# Autodesk Inventor assembly: OBG-Elektronik
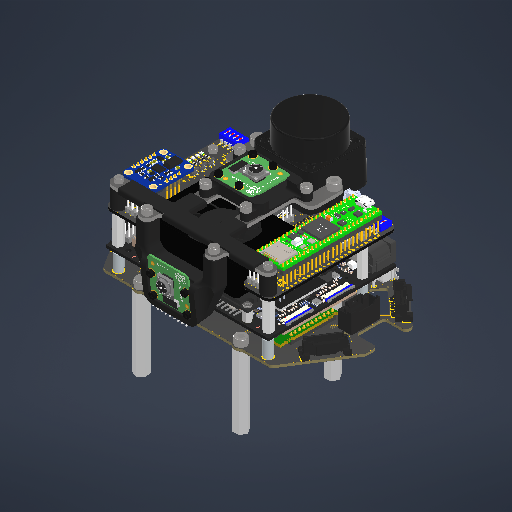
[picture p0: Inventor's stored thumbnail of the model, 512x512]
Saved by Autodesk Inventor 2025.2 (Build 292293000, 293)
## iProperties
Created: 2024-11-26
Part Number: OBG-Elektronik
Document SubType Name: Assembly
Designer: Fabian
Author: Fabian
## Documents named in this file (19)
- C:\Users\Faabs\Desktop\HBG v2025\Oberbaugruppen\OBG-Elektronik\OBG-Elektronik.iam
- C:\Users\Faabs\Desktop\HBG v2025\Oberbaugruppen\OBG-Elektronik\Bauteile\Abstandsbolzen 45mm.ipt
- C:\Users\Faabs\Desktop\HBG v2025\Oberbaugruppen\OBG-Elektronik\Bauteile\Jetson Orin Nano\Jetson Orin Nano.iam
- C:\Users\Faabs\Desktop\HBG v2025\Oberbaugruppen\OBG-Elektronik\Bauteile\Abstandsbolzen 17mm.ipt
- C:\Users\Faabs\Desktop\HBG v2025\Oberbaugruppen\OBG-Elektronik\Bauteile\360° LiDAR\360° LiDAR.iam
- C:\Users\Faabs\Desktop\HBG v2025\Verbindungselemente\DIN 912\DIN 912 - M4 x 0,7 x 8 x 6,25.ipt
- C:\Users\Faabs\Desktop\HBG v2025\Verbindungselemente\DIN 912\DIN 912 - M2,5 x 0,45 x 8 x 6,875.ipt
- C:\Users\Faabs\Desktop\HBG v2025\Oberbaugruppen\OBG-Elektronik\Bauteile\Trägerblech.ipt
- C:\Users\Faabs\Desktop\HBG v2025\Oberbaugruppen\OBG-Elektronik\Bauteile\Kamera.ipt
- C:\Users\Faabs\Desktop\HBG v2025\Oberbaugruppen\OBG-Elektronik\Bauteile\Kamerahalterung oben.ipt
- C:\Users\Faabs\Desktop\HBG v2025\Verbindungselemente\DIN 912\DIN 912 - M3 x 0,5 x 5 x 3,75.ipt
- C:\Users\Faabs\Desktop\HBG v2025\Oberbaugruppen\OBG-Elektronik\Bauteile\Abstandshalter 11mm.ipt
- C:\Users\Faabs\Desktop\HBG v2025\Oberbaugruppen\OBG-Elektronik\Bauteile\Abstandshalter 7,4mm.ipt
- C:\Users\Faabs\Desktop\HBG v2025\Verbindungselemente\DIN 912\DIN 912 - M4 x 0,7 x 16 x 14,25.ipt
- C:\Users\Faabs\Desktop\HBG v2025\Platinen\Steuerplatine\Steuerplatine\Steuerplatine.iam
- C:\Users\Faabs\Desktop\HBG v2025\Platinen\Hauptplatine\HauptplatineV2\HauptplatineV2.iam
- C:\Users\Faabs\Desktop\HBG v2025\Oberbaugruppen\OBG-Elektronik\Bauteile\Spiegelflächenabdeckung.ipt
- C:\Users\Faabs\Desktop\HBG v2025\Oberbaugruppen\OBG-Elektronik\Bauteile\Kamerahalterung vorne.ipt
- C:\Users\Faabs\Desktop\HBG v2025\Verbindungselemente\DIN 912\DIN 912 - M2 x 0,4 x 4 x 3.ipt
## Components (46 placed, 18 different names)
1. Jetson Orin Nano:1 [sub-assembly] — Passend:14, Passend:15, Passend:16, Passend:17, Passend:18, Passend:19, Passend:20, Passend:21, Passend:76
2. Steuerplatine:1 [sub-assembly] — Einfügen:27, Einfügen:29, Einfügen:30, Einfügen:35, Einfügen:36, Passend:79, Passend:80, Passend:82, Passend:83
3. HauptplatineV2:1 [sub-assembly] — Passend:64, Fluchtend:1, Passend:74, Passend:75, Passend:76, Passend:106, Passend:107, Passend:108, Passend:109, Passend:110, Passend:111, Passend:112, Passend:113, Einfügen:44, Einfügen:45, Einfügen:46, Einfügen:47
4. 360° LiDAR:1 [sub-assembly] — Passend:48, Passend:49, Passend:50, Passend:51, Einfügen:29, Einfügen:30
5. DIN 912 - ersetzt durch DIN EN ISO 4762 M2 x 4:8 — Einfügen:52
6. DIN 912 - ersetzt durch DIN EN ISO 4762 M2 x 4:7 — Einfügen:53
7. DIN 912 - ersetzt durch DIN EN ISO 4762 M2 x 4:6 — Einfügen:54
8. DIN 912 - ersetzt durch DIN EN ISO 4762 M2 x 4:5 — Einfügen:55
9. DIN 912 - ersetzt durch DIN EN ISO 4762 M2 x 4:4 — Einfügen:51
10. DIN 912 - ersetzt durch DIN EN ISO 4762 M2 x 4:3 — Einfügen:49
11. DIN 912 - ersetzt durch DIN EN ISO 4762 M2 x 4:2 — Einfügen:50
12. DIN 912 - ersetzt durch DIN EN ISO 4762 M2 x 4:1 — Einfügen:48
13. DIN 912 - ersetzt durch DIN EN ISO 4762 M3 x 5:6 — Einfügen:42
14. DIN 912 - ersetzt durch DIN EN ISO 4762 M3 x 5:5 — Einfügen:41, Passend:102
15. DIN 912 - ersetzt durch DIN EN ISO 4762 M4 x 16:2 — Einfügen:18
16. DIN 912 - ersetzt durch DIN EN ISO 4762 M4 x 16:1 — Einfügen:17
17. DIN 912 - ersetzt durch DIN EN ISO 4762 M3 x 5:4 — Einfügen:11
18. DIN 912 - ersetzt durch DIN EN ISO 4762 M3 x 5:3 — Einfügen:12
19. DIN 912 - ersetzt durch DIN EN ISO 4762 M3 x 5:2 — Einfügen:13
20. DIN 912 - ersetzt durch DIN EN ISO 4762 M3 x 5:1 — Einfügen:14
21. DIN 912 - ersetzt durch DIN EN ISO 4762 M4 x 8:1 — Einfügen:44
22. DIN 912 - ersetzt durch DIN EN ISO 4762 M4 x 8:2 — Einfügen:45
23. DIN 912 - ersetzt durch DIN EN ISO 4762 M4 x 8:3 — Einfügen:47
24. DIN 912 - ersetzt durch DIN EN ISO 4762 M4 x 8:4 — Einfügen:46
25. DIN 912 - ersetzt durch DIN EN ISO 4762 M2,5 x 8:1 — Einfügen:39
26. DIN 912 - ersetzt durch DIN EN ISO 4762 M2,5 x 8:2 — Einfügen:35, Passend:81
27. DIN 912 - ersetzt durch DIN EN ISO 4762 M2,5 x 8:3 — Einfügen:40
28. DIN 912 - ersetzt durch DIN EN ISO 4762 M2,5 x 8:4 — Einfügen:36
29. Abstandshalter 11mm:1 — Passend:82, Passend:83, Passend:85
30. Abstandshalter 11mm:2 — Einfügen:27, Passend:84
31. Abstandshalter 7,4mm:1 — Passend:49, Passend:50, Passend:63
32. Abstandshalter 7,4mm:2 — Passend:48, Passend:51
33. Abstandsbolzen 45mm:1 — Passend:108, Passend:113
34. Abstandsbolzen 45mm:2 — Passend:109, Passend:110
35. Abstandsbolzen 45mm:3 — Passend:106, Passend:111, Passend:114
36. Abstandsbolzen 45mm:4 — Passend:107, Passend:112
37. Abstandsbolzen 17mm:1 — Passend:14, Passend:21, Passend:79, Passend:80
38. Abstandsbolzen 17mm:2 — Passend:15, Passend:18, Passend:75
39. Abstandsbolzen 17mm:3 — Passend:16, Passend:20, Passend:74
40. Abstandsbolzen 17mm:4 — Passend:17, Passend:19, Passend:81
41. Kamera:3 — Passend:103, Passend:104, Passend:105, Einfügen:52, Einfügen:53, Einfügen:54, Einfügen:55
42. Kamerahalterung vorne:1 — Einfügen:43, Passend:102, Passend:103, Passend:104, Passend:105
43. Spiegelflächenabdeckung:1 — Passend:98, Passend:99, Passend:100
44. Trägerblech:1 — Passend:38, Einfügen:17, Einfügen:18, Passend:63, Einfügen:37, Einfügen:38, Passend:84, Passend:85, Einfügen:39, Einfügen:40, Passend:98, Passend:99, Passend:100, Einfügen:41, Einfügen:42, Einfügen:43
45. Kamera:1 — Passend:39, Passend:40, Passend:41, Einfügen:48, Einfügen:49, Einfügen:50, Einfügen:51
46. Kamerahalterung oben:1 — Passend:38, Passend:39, Passend:40, Passend:41, Einfügen:11, Einfügen:12, Einfügen:13, Einfügen:14, Einfügen:37, Einfügen:38
## Relationships (75: Mate 44, Insert 30, Flush 1)
- Passend:14 [Mate]: Jetson Orin Nano:1 ↔ Abstandsbolzen 17mm:1
- Passend:15 [Mate]: Jetson Orin Nano:1 ↔ Abstandsbolzen 17mm:2
- Passend:16 [Mate]: Jetson Orin Nano:1 ↔ Abstandsbolzen 17mm:3
- Passend:17 [Mate]: Jetson Orin Nano:1 ↔ Abstandsbolzen 17mm:4
- Passend:18 [Mate]: Jetson Orin Nano:1 ↔ Abstandsbolzen 17mm:2
- Passend:19 [Mate]: Jetson Orin Nano:1 ↔ Abstandsbolzen 17mm:4
- Passend:20 [Mate]: Jetson Orin Nano:1 ↔ Abstandsbolzen 17mm:3
- Passend:21 [Mate]: Jetson Orin Nano:1 ↔ Abstandsbolzen 17mm:1
- Passend:38 [Mate]: Trägerblech:1 ↔ Kamerahalterung oben:1
- Passend:39 [Mate]: Kamera:1 ↔ Kamerahalterung oben:1
- Passend:40 [Mate]: Kamera:1 ↔ Kamerahalterung oben:1
- Passend:41 [Mate]: Kamera:1 ↔ Kamerahalterung oben:1
- Einfügen:11 [Insert]: DIN 912 - ersetzt durch DIN EN ISO 4762 M3 x 5:4 ↔ Kamerahalterung oben:1
- Einfügen:12 [Insert]: DIN 912 - ersetzt durch DIN EN ISO 4762 M3 x 5:3 ↔ Kamerahalterung oben:1
- Einfügen:13 [Insert]: DIN 912 - ersetzt durch DIN EN ISO 4762 M3 x 5:2 ↔ Kamerahalterung oben:1
- Einfügen:14 [Insert]: DIN 912 - ersetzt durch DIN EN ISO 4762 M3 x 5:1 ↔ Kamerahalterung oben:1
- Passend:48 [Mate]: 360° LiDAR:1 ↔ Abstandshalter 7,4mm:2
- Passend:49 [Mate]: 360° LiDAR:1 ↔ Abstandshalter 7,4mm:1
- Passend:50 [Mate]: 360° LiDAR:1 ↔ Abstandshalter 7,4mm:1
- Passend:51 [Mate]: 360° LiDAR:1 ↔ Abstandshalter 7,4mm:2
- Einfügen:17 [Insert]: DIN 912 - ersetzt durch DIN EN ISO 4762 M4 x 16:1 ↔ Trägerblech:1
- Einfügen:18 [Insert]: DIN 912 - ersetzt durch DIN EN ISO 4762 M4 x 16:2 ↔ Trägerblech:1
- Einfügen:27 [Insert]: Steuerplatine:1 ↔ Abstandshalter 11mm:2
- Einfügen:29 [Insert]: Steuerplatine:1 ↔ 360° LiDAR:1
- Einfügen:30 [Insert]: Steuerplatine:1 ↔ 360° LiDAR:1
- Passend:63 [Mate]: Abstandshalter 7,4mm:1 ↔ Trägerblech:1
- Passend:64 [Mate]: HauptplatineV2:1
- Fluchtend:1 [Flush]: HauptplatineV2:1
- Einfügen:35 [Insert]: Steuerplatine:1 ↔ DIN 912 - ersetzt durch DIN EN ISO 4762 M2,5 x 8:2
- Einfügen:36 [Insert]: Steuerplatine:1 ↔ DIN 912 - ersetzt durch DIN EN ISO 4762 M2,5 x 8:4
- Passend:74 [Mate]: HauptplatineV2:1 ↔ Abstandsbolzen 17mm:3
- Passend:75 [Mate]: HauptplatineV2:1 ↔ Abstandsbolzen 17mm:2
- Passend:76 [Mate] (2 mm): Jetson Orin Nano:1 ↔ HauptplatineV2:1
- Einfügen:37 [Insert]: Trägerblech:1 ↔ Kamerahalterung oben:1
- Einfügen:38 [Insert]: Trägerblech:1 ↔ Kamerahalterung oben:1
- Passend:79 [Mate] (2 mm): Steuerplatine:1 ↔ Abstandsbolzen 17mm:1
- Passend:80 [Mate]: Steuerplatine:1 ↔ Abstandsbolzen 17mm:1
- Passend:81 [Mate]: DIN 912 - ersetzt durch DIN EN ISO 4762 M2,5 x 8:2 ↔ Abstandsbolzen 17mm:4
- Passend:82 [Mate]: Steuerplatine:1 ↔ Abstandshalter 11mm:1
- Passend:83 [Mate]: Steuerplatine:1 ↔ Abstandshalter 11mm:1
- Passend:84 [Mate]: Abstandshalter 11mm:2 ↔ Trägerblech:1
- Passend:85 [Mate]: Abstandshalter 11mm:1 ↔ Trägerblech:1
- Einfügen:39 [Insert]: DIN 912 - ersetzt durch DIN EN ISO 4762 M2,5 x 8:1 ↔ Trägerblech:1
- Einfügen:40 [Insert]: DIN 912 - ersetzt durch DIN EN ISO 4762 M2,5 x 8:3 ↔ Trägerblech:1
- Passend:98 [Mate]: Spiegelflächenabdeckung:1 ↔ Trägerblech:1
- Passend:99 [Mate]: Spiegelflächenabdeckung:1 ↔ Trägerblech:1
- Passend:100 [Mate]: Spiegelflächenabdeckung:1 ↔ Trägerblech:1
- Einfügen:41 [Insert]: DIN 912 - ersetzt durch DIN EN ISO 4762 M3 x 5:5 ↔ Trägerblech:1
- Einfügen:42 [Insert]: DIN 912 - ersetzt durch DIN EN ISO 4762 M3 x 5:6 ↔ Trägerblech:1
- Einfügen:43 [Insert]: Kamerahalterung vorne:1 ↔ Trägerblech:1
- Passend:102 [Mate]: DIN 912 - ersetzt durch DIN EN ISO 4762 M3 x 5:5 ↔ Kamerahalterung vorne:1
- Passend:103 [Mate]: Kamera:3 ↔ Kamerahalterung vorne:1
- Passend:104 [Mate]: Kamera:3 ↔ Kamerahalterung vorne:1
- Passend:105 [Mate]: Kamera:3 ↔ Kamerahalterung vorne:1
- Passend:106 [Mate]: HauptplatineV2:1 ↔ Abstandsbolzen 45mm:3
- Passend:107 [Mate]: HauptplatineV2:1 ↔ Abstandsbolzen 45mm:4
- Passend:108 [Mate]: HauptplatineV2:1 ↔ Abstandsbolzen 45mm:1
- Passend:109 [Mate]: HauptplatineV2:1 ↔ Abstandsbolzen 45mm:2
- Passend:110 [Mate]: HauptplatineV2:1 ↔ Abstandsbolzen 45mm:2
- Passend:111 [Mate]: HauptplatineV2:1 ↔ Abstandsbolzen 45mm:3
- Passend:112 [Mate]: HauptplatineV2:1 ↔ Abstandsbolzen 45mm:4
- Passend:113 [Mate]: HauptplatineV2:1 ↔ Abstandsbolzen 45mm:1
- Einfügen:44 [Insert]: HauptplatineV2:1 ↔ DIN 912 - ersetzt durch DIN EN ISO 4762 M4 x 8:1
- Einfügen:45 [Insert]: HauptplatineV2:1 ↔ DIN 912 - ersetzt durch DIN EN ISO 4762 M4 x 8:2
- Einfügen:46 [Insert]: HauptplatineV2:1 ↔ DIN 912 - ersetzt durch DIN EN ISO 4762 M4 x 8:4
- Einfügen:47 [Insert]: HauptplatineV2:1 ↔ DIN 912 - ersetzt durch DIN EN ISO 4762 M4 x 8:3
- Passend:114 [Mate]: Abstandsbolzen 45mm:3
- Einfügen:48 [Insert]: DIN 912 - ersetzt durch DIN EN ISO 4762 M2 x 4:1 ↔ Kamera:1
- Einfügen:49 [Insert]: DIN 912 - ersetzt durch DIN EN ISO 4762 M2 x 4:3 ↔ Kamera:1
- Einfügen:50 [Insert]: DIN 912 - ersetzt durch DIN EN ISO 4762 M2 x 4:2 ↔ Kamera:1
- Einfügen:51 [Insert]: DIN 912 - ersetzt durch DIN EN ISO 4762 M2 x 4:4 ↔ Kamera:1
- Einfügen:52 [Insert]: DIN 912 - ersetzt durch DIN EN ISO 4762 M2 x 4:8 ↔ Kamera:3
- Einfügen:53 [Insert]: DIN 912 - ersetzt durch DIN EN ISO 4762 M2 x 4:7 ↔ Kamera:3
- Einfügen:54 [Insert]: DIN 912 - ersetzt durch DIN EN ISO 4762 M2 x 4:6 ↔ Kamera:3
- Einfügen:55 [Insert]: DIN 912 - ersetzt durch DIN EN ISO 4762 M2 x 4:5 ↔ Kamera:3
